# Autodesk Inventor assembly: Full Octopus
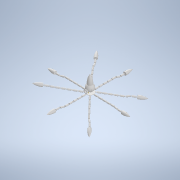
[picture p0: Inventor's stored thumbnail of the model, 180x180]
Saved by Autodesk Inventor 2022 (Build 260153000, 153)
## iProperties
Created: 2020-07-11
Part Number: Full Octopus
Document SubType Name: Assembly
Designer: saipr
Author: saipr
## Documents named in this file (3)
- C:\Users\saipr\Desktop\Autodesk 2022\Builds\Parts\Full Octopus.iam
- C:\Users\saipr\Desktop\Autodesk 2022\Builds\Parts\octopus.ipt
- C:\Users\saipr\Desktop\Autodesk 2022\Builds\Parts\Tentacle Full.iam
## Components (9 placed, 2 different names)
1. octopus:1 — Mate:1, Mate:2, Mate:3, Mate:4, Mate:5, Mate:6, Mate:7, Mate:8
2. Tentacle Full:1 [sub-assembly] — Mate:2
3. Tentacle Full:2 [sub-assembly] — Mate:3
4. Tentacle Full:3 [sub-assembly] — Mate:4
5. Tentacle Full:4 [sub-assembly] — Mate:1
6. Tentacle Full:5 [sub-assembly] — Mate:5
7. Tentacle Full:6 [sub-assembly] — Mate:7
8. Tentacle Full:7 [sub-assembly] — Mate:8
9. Tentacle Full:8 [sub-assembly] — Mate:6
## Relationships (8: Mate 8)
- Mate:1: octopus:1 ↔ Tentacle Full:4
- Mate:2: octopus:1 ↔ Tentacle Full:1
- Mate:3: octopus:1 ↔ Tentacle Full:2
- Mate:4: octopus:1 ↔ Tentacle Full:3
- Mate:5: octopus:1 ↔ Tentacle Full:5
- Mate:6: octopus:1 ↔ Tentacle Full:8
- Mate:7: octopus:1 ↔ Tentacle Full:6
- Mate:8: octopus:1 ↔ Tentacle Full:7
